# Autodesk Inventor assembly: 射出機構
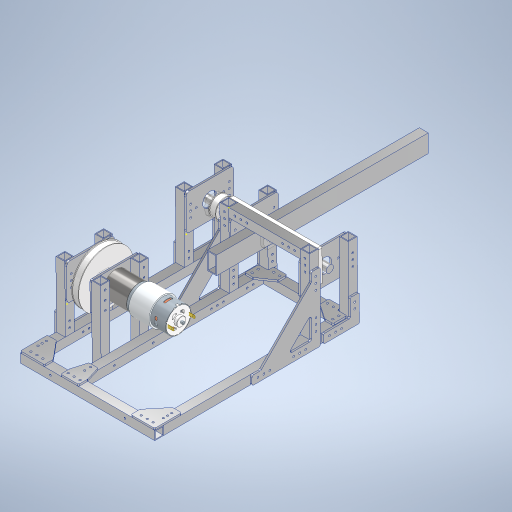
[picture p0: Inventor's stored thumbnail of the model, 512x512]
Saved by Autodesk Inventor 2023 (Build 270158000, 158)
## iProperties
Created: 2022-04-24
Part Number: 射出機構
Document SubType Name: Assembly
Designer: yuta
Mass: 1983.22 g
Surface Area: 5502.15 cm^2
Volume: 620.531 cm^3
Density: 3.19601 g/cm^3
Author: yuta
## Documents named in this file (8)
- C:\Users\yuta\Documents\NHK\射出機構.iam
- C:\Users\yuta\Documents\NHK\射出_骨組み.iam
- C:\Users\yuta\Documents\NHK\射出_モーター.iam
- C:\Users\yuta\Documents\NHK\射出_ベアリング1.iam
- C:\Users\yuta\Documents\NHK\射出_上部.iam
- C:\Users\yuta\Documents\NHK\射出_本体.iam
- C:\Users\yuta\Documents\NHK\射出_軸.iam
- C:\Users\yuta\Documents\NHK\射出_腕.iam
## Components (8 placed, 7 different names)
1. 射出_骨組み:1 [sub-assembly] — メイト:1, メイト:2, メイト:3, メイト:4, メイト:5, メイト:6, メイト:7, メイト:29, メイト:30, メイト:31, メイト:32, メイト:33, メイト:34, メイト:35, メイト:36, メイト:37, メイト:38, メイト:39, メイト:40
2. 射出_モーター:1 [sub-assembly] — メイト:1, メイト:2, メイト:3, メイト:12, メイト:13
3. 射出_ベアリング1:1 [sub-assembly] — メイト:4, メイト:5, メイト:6, メイト:7
4. 射出_本体:1 [sub-assembly] — メイト:12, メイト:13, フラッシュ:1
5. 射出_上部:1 [sub-assembly] — メイト:29, メイト:30, メイト:31, メイト:32, メイト:33, メイト:34, メイト:35, メイト:36, メイト:37, メイト:41, メイト:43
6. 射出_ベアリング1:2 [sub-assembly] — メイト:38, メイト:39, メイト:40
7. 射出_軸:1 [sub-assembly] — メイト:41, フラッシュ:1, メイト:42
8. 射出_腕:1 [sub-assembly] — メイト:42, メイト:43
## Relationships (25: Mate 24, Flush 1)
- メイト:1 [Mate]: 射出_骨組み:1 ↔ 射出_モーター:1
- メイト:2 [Mate]: 射出_骨組み:1 ↔ 射出_モーター:1
- メイト:3 [Mate]: 射出_骨組み:1 ↔ 射出_モーター:1
- メイト:4 [Mate]: 射出_骨組み:1 ↔ 射出_ベアリング1:1
- メイト:5 [Mate]: 射出_骨組み:1 ↔ 射出_ベアリング1:1
- メイト:6 [Mate]: 射出_骨組み:1 ↔ 射出_ベアリング1:1
- メイト:7 [Mate]: 射出_骨組み:1 ↔ 射出_ベアリング1:1
- メイト:12 [Mate]: 射出_モーター:1 ↔ 射出_本体:1
- メイト:13 [Mate]: 射出_モーター:1 ↔ 射出_本体:1
- メイト:29 [Mate]: 射出_骨組み:1 ↔ 射出_上部:1
- メイト:30 [Mate]: 射出_骨組み:1 ↔ 射出_上部:1
- メイト:31 [Mate]: 射出_骨組み:1 ↔ 射出_上部:1
- メイト:32 [Mate]: 射出_骨組み:1 ↔ 射出_上部:1
- メイト:33 [Mate]: 射出_骨組み:1 ↔ 射出_上部:1
- メイト:34 [Mate]: 射出_骨組み:1 ↔ 射出_上部:1
- メイト:35 [Mate]: 射出_骨組み:1 ↔ 射出_上部:1
- メイト:36 [Mate]: 射出_骨組み:1 ↔ 射出_上部:1
- メイト:37 [Mate]: 射出_骨組み:1 ↔ 射出_上部:1
- メイト:38 [Mate]: 射出_骨組み:1 ↔ 射出_ベアリング1:2
- メイト:39 [Mate]: 射出_骨組み:1 ↔ 射出_ベアリング1:2
- メイト:40 [Mate]: 射出_骨組み:1 ↔ 射出_ベアリング1:2
- メイト:41 [Mate]: 射出_上部:1 ↔ 射出_軸:1
- フラッシュ:1 [Flush]: 射出_本体:1 ↔ 射出_軸:1
- メイト:42 [Mate]: 射出_軸:1 ↔ 射出_腕:1
- メイト:43 [Mate] (5 mm): 射出_上部:1 ↔ 射出_腕:1
